# Autodesk Inventor assembly: HipLeftExact
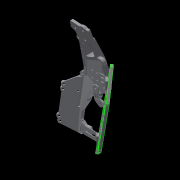
[picture p0: Inventor's stored thumbnail of the model, 180x180]
Saved by Autodesk Inventor 2015 (Build 190159000, 159)
## iProperties
Created: 2014-09-01
Part Number: HipLeftExact
Document SubType Name: Assembly
Designer: Inventor
Mass: 809.946 g
Surface Area: 1272.46 cm^2
Volume: 359.464 cm^3
Density: 2.2532 g/cm^3
Author: Inventor
## Documents named in this file (6)
- G:\Exo\Models\3D\HipLeft.iam
- G:\Exo\Models\3D\HipLeft.ipt
- G:\Exo\Models\3D\HipTopConnectorLeft.ipt
- G:\Exo\Models\3D\HipBottomConnectorLeft.ipt
- G:\Exo\Models\3D\HipShockPlateLeft.ipt
- G:\Exo\Models\3D\HipPistonConnectorLeft.ipt
## Components (5 placed, 5 different names)
1. HipLeft:1 — Angle:1, Mate:7, Mate:8, Mate:9, Mate:10, Mate:11, Angle:2, Mate:16, Mate:17, Flush:2
2. HipTopConnectorLeft:1 — Angle:1, Angle:3, Mate:14, Mate:15, Mate:16, Mate:17, Flush:2
3. HipBottomConnectorLeft:1 — Mate:9, Mate:10, Mate:11, Angle:2, Flush:1
4. HipShockPlateLeft:1 — Angle:3, Mate:14, Mate:15, Flush:1
5. HipPistonConnectorLeft:1 — Mate:7, Mate:8
## Relationships (14: Mate 9, Angle 3, Flush 2)
- Angle:1 (180 deg): HipLeft:1 ↔ HipTopConnectorLeft:1
- Mate:7: HipLeft:1 ↔ HipPistonConnectorLeft:1
- Mate:8: HipLeft:1 ↔ HipPistonConnectorLeft:1
- Mate:9: HipLeft:1 ↔ HipBottomConnectorLeft:1
- Mate:10: HipLeft:1 ↔ HipBottomConnectorLeft:1
- Mate:11: HipLeft:1 ↔ HipBottomConnectorLeft:1
- Angle:2 (0 deg): HipLeft:1 ↔ HipBottomConnectorLeft:1
- Angle:3 (180 deg): HipTopConnectorLeft:1 ↔ HipShockPlateLeft:1
- Mate:14: HipTopConnectorLeft:1 ↔ HipShockPlateLeft:1
- Mate:15: HipTopConnectorLeft:1 ↔ HipShockPlateLeft:1
- Mate:16: HipLeft:1 ↔ HipTopConnectorLeft:1
- Mate:17: HipLeft:1 ↔ HipTopConnectorLeft:1
- Flush:1: HipBottomConnectorLeft:1 ↔ HipShockPlateLeft:1
- Flush:2: HipLeft:1 ↔ HipTopConnectorLeft:1
